# Autodesk Inventor assembly: dome one terminal
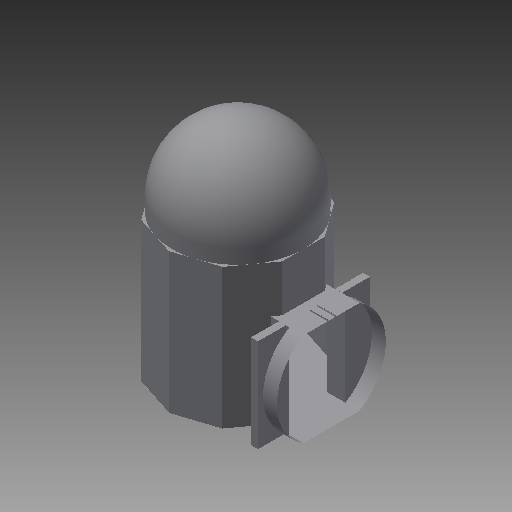
[picture p0: Inventor's stored thumbnail of the model, 512x512]
Saved by Autodesk Inventor 2017 (Build 210142000, 142)
## iProperties
Created: 2018-04-12
Part Number: dome one terminal
Document SubType Name: Assembly
Designer: Braxton
Author: Braxton
## Documents named in this file (3)
- E:\School\Game develpment\geoscape\done\single wall\rooms  (one wall)\assembly\dome one terminal.iam
- E:\School\Game develpment\geoscape\done\single wall\rooms  (one wall)\dome one terminal  (one wall).ipt
- E:\School\Game develpment\geoscape\done\doors\double door.ipt
## Components (3 placed, 2 different names)
1. dome one terminal  (one wall):1 — Mate:3, Mate:4, Mate:5, Mate:6, Mate:7, Mate:8
2. double door:1 — Mate:3, Mate:6, Mate:7
3. double door:2 — Mate:4, Mate:5, Mate:8
## Relationships (6: Mate 6)
- Mate:3: dome one terminal  (one wall):1 ↔ double door:1
- Mate:4: dome one terminal  (one wall):1 ↔ double door:2
- Mate:5: dome one terminal  (one wall):1 ↔ double door:2
- Mate:6: dome one terminal  (one wall):1 ↔ double door:1
- Mate:7: dome one terminal  (one wall):1 ↔ double door:1
- Mate:8: dome one terminal  (one wall):1 ↔ double door:2
